# Autodesk Inventor assembly: robot_assembly
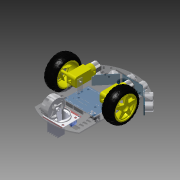
[picture p0: Inventor's stored thumbnail of the model, 180x180]
Saved by Autodesk Inventor 2015 (Build 190159000, 159)
## iProperties
Created: 2021-07-12
Part Number: robot_assembly
Document SubType Name: Assembly
Designer: Captain
Author: Captain
## Documents named in this file (8)
- C:\Users\Captain\Desktop\Project Folder\Software\Qzadok_Auto-robot\3D Model\robot_assembly.iam
- C:\Users\Captain\Desktop\Project Folder\Software\Qzadok_Auto-robot\3D Model\chassis.ipt
- C:\Users\Captain\Desktop\Project Folder\Software\Qzadok_Auto-robot\3D Model\wheel.ipt
- C:\Users\Captain\Desktop\Project Folder\Software\Qzadok_Auto-robot\3D Model\motor_dc.ipt
- C:\Users\Captain\Desktop\Project Folder\Software\Qzadok_Auto-robot\3D Model\castor_wheel.iam
- C:\Users\Captain\Desktop\Project Folder\Software\Qzadok_Auto-robot\3D Model\motor_driver.ipt
- C:\Users\Captain\Desktop\Project Folder\Software\Qzadok_Auto-robot\3D Model\arduino_uno.ipt
- C:\Users\Captain\Desktop\Project Folder\Software\Qzadok_Auto-robot\3D Model\ultra_sonic_sensor.ipt
## Components (11 placed, 7 different names)
1. chassis:1 — Mate:1, Angle:1, Mate:2, Angle:2, Angle:3, Mate:3, Angle:4, Angle:6, Angle:8, Angle:9, Mate:4, Mate:5, Angle:10, Mate:6, Angle:11, Mate:7
2. wheel:1 — Mate:1, Insert:1, Angle:7, Angle:8
3. motor_dc:1 — Insert:1, Angle:1
4. wheel:2 — Mate:2, Insert:2, Angle:3, Angle:7
5. motor_dc:2 — Insert:2, Angle:2
6. castor_wheel:1 [sub-assembly] — Mate:3, Angle:4, Angle:5
7. motor_driver:1 — Angle:5, Angle:6
8. arduino_uno:1 — Angle:9, Mate:4
9. ultra_sonic_sensor:1 — Mate:5, Angle:10
10. ultra_sonic_sensor:2 — Mate:7
11. ultra_sonic_sensor:3 — Mate:6, Angle:11
## Relationships (20: Angle 11, Mate 7, Insert 2)
- Mate:1: chassis:1 ↔ wheel:1
- Insert:1 (-1.5 mm): wheel:1 ↔ motor_dc:1
- Angle:1 (0 deg): chassis:1 ↔ motor_dc:1
- Mate:2: chassis:1 ↔ wheel:2
- Insert:2 (-1.5 mm): wheel:2 ↔ motor_dc:2
- Angle:2 (180 deg): chassis:1 ↔ motor_dc:2
- Angle:3 (0 deg): chassis:1 ↔ wheel:2
- Mate:3: chassis:1 ↔ castor_wheel:1
- Angle:4 (180 deg): chassis:1 ↔ castor_wheel:1
- Angle:5 (180 deg): castor_wheel:1 ↔ motor_driver:1
- Angle:6 (180 deg): chassis:1 ↔ motor_driver:1
- Angle:7 (0 deg): wheel:1 ↔ wheel:2
- Angle:8 (90 deg): chassis:1 ↔ wheel:1
- Angle:9 (180 deg): chassis:1 ↔ arduino_uno:1
- Mate:4: chassis:1 ↔ arduino_uno:1
- Mate:5: chassis:1 ↔ ultra_sonic_sensor:1
- Angle:10 (220 deg): chassis:1 ↔ ultra_sonic_sensor:1
- Mate:6: chassis:1 ↔ ultra_sonic_sensor:3
- Angle:11 (315 deg): chassis:1 ↔ ultra_sonic_sensor:3
- Mate:7: chassis:1 ↔ ultra_sonic_sensor:2
